# Autodesk Inventor assembly: Tube_ObjLens+RaspiCam
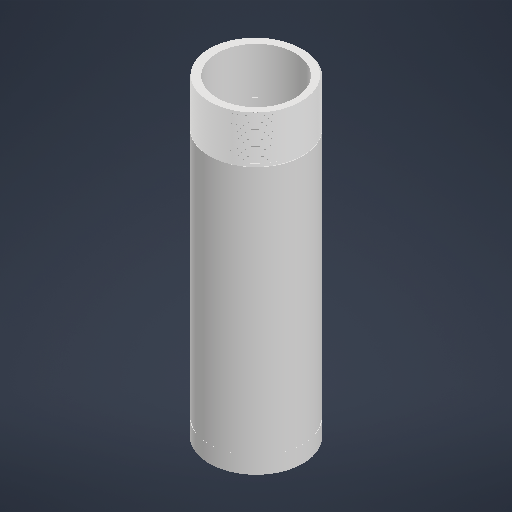
[picture p0: Inventor's stored thumbnail of the model, 512x512]
Saved by Autodesk Inventor 2026.2 (Build 302298000, 298)
## iProperties
Created: 2026-03-11
Part Number: Tube_ObjLens+RaspiCam
Document SubType Name: Assembly
Designer: Alvin
Author: Alvin
## Documents named in this file (4)
- C:\Users\Alvin\OneDrive\Documents\Inventor\NCKU_Automation_Incubator_Microscope\Tube_ObjLens+RaspiCam.iam
- C:\Users\Alvin\OneDrive\Documents\Inventor\NCKU_Automation_Incubator_Microscope\objlensmount_part-1.ipt
- C:\Users\Alvin\OneDrive\Documents\Inventor\NCKU_Automation_Incubator_Microscope\objlensmount_part-2.ipt
- C:\Users\Alvin\OneDrive\Documents\Inventor\NCKU_Automation_Incubator_Microscope\objlensmount_part-3.ipt
## Components (3 placed, 3 different names)
1. objlensmount_part-1:1 — Mate:1, Mate:2, Mate:3, Mate:4
2. objlensmount_part-2:1 — Mate:1, Mate:2
3. objlensmount_part-3:1 — Mate:3, Mate:4
## Relationships (7: Mate 4, Angle 3)
- Mate:1: objlensmount_part-1:1 ↔ objlensmount_part-2:1
- Mate:2: objlensmount_part-1:1 ↔ objlensmount_part-2:1
- Mate:3: objlensmount_part-1:1 ↔ objlensmount_part-3:1
- Mate:4: objlensmount_part-1:1 ↔ objlensmount_part-3:1
- Angle:1 (0 deg)
- Angle:2 (0 deg)
- Angle:3 (0 deg)
